# Autodesk Inventor assembly: Gripper
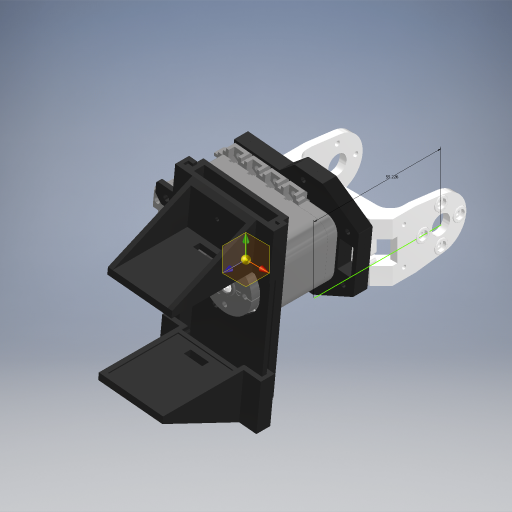
[picture p0: Inventor's stored thumbnail of the model, 512x512]
Saved by Autodesk Inventor 2024 (Build 280153000, 153)
## iProperties
Created: 2023-09-03
Part Number: Gripper
Document SubType Name: Assembly
Designer: arrusr01
Mass: 128.702 g
Surface Area: 490.072 cm^2
Volume: 78.3197 cm^3
Density: 1.64329 g/cm^3
Author: arrusr01
## Documents named in this file (6)
- C:\Users\arrusr01\OneDrive\Semestres\Inventor\Adaptable\Gripper.iam
- C:\Users\arrusr01\OneDrive\Semestres\Inventor\Adaptable\FP04-F2\FP04-F2.ipt
- C:\Users\arrusr01\OneDrive\Semestres\Inventor\interbotix-phantomx-reactor-robot-arm-kit-1.snapshot.1\InterbotiX PhantomX Reactor Robot Arm Kit\Wrist Top.ipt
- C:\Users\arrusr01\OneDrive\Semestres\Inventor\Adaptable\AX-12\AX-12.ipt
- C:\Users\arrusr01\OneDrive\Semestres\Inventor\interbotix-phantomx-reactor-robot-arm-kit-1.snapshot.1\InterbotiX PhantomX Reactor Robot Arm Kit\rails v1.ipt
- C:\Users\arrusr01\OneDrive\Semestres\Inventor\interbotix-phantomx-reactor-robot-arm-kit-1.snapshot.1\InterbotiX PhantomX Reactor Robot Arm Kit\RightFinger v2.ipt
## Components (7 placed, 5 different names)
1. FP04-F2:1 — Mate:1, Insert:1
2. Wrist Top:1 — Insert:2, Flush:1, Mate:2, Mate:3
3. Wrist Top:3 — Mate:1, Insert:1, Insert:2, Flush:1, Mate:4
4. AX-12:1 — Mate:2, Mate:3, Mate:4, Mate:5, Insert:3, Mate:6
5. rails v1:1 — Mate:5, Insert:3, Mate:6, Mate:7, Mate:8, Mate:9, Mate:10
6. RightFinger v2:1 — Mate:9, Mate:10
7. RightFinger v2:2 — Mate:7, Mate:8
## Relationships (14: Mate 10, Insert 3, Flush 1)
- Mate:1: FP04-F2:1 ↔ Wrist Top:3
- Insert:1: FP04-F2:1 ↔ Wrist Top:3
- Insert:2: Wrist Top:1 ↔ Wrist Top:3
- Flush:1: Wrist Top:1 ↔ Wrist Top:3
- Mate:2: Wrist Top:1 ↔ AX-12:1
- Mate:3: Wrist Top:1 ↔ AX-12:1
- Mate:4: Wrist Top:3 ↔ AX-12:1
- Mate:5: AX-12:1 ↔ rails v1:1
- Insert:3: AX-12:1 ↔ rails v1:1
- Mate:6: AX-12:1 ↔ rails v1:1
- Mate:7: rails v1:1 ↔ RightFinger v2:2
- Mate:8: rails v1:1 ↔ RightFinger v2:2
- Mate:9: rails v1:1 ↔ RightFinger v2:1
- Mate:10: rails v1:1 ↔ RightFinger v2:1
